# Autodesk Inventor assembly: elric20
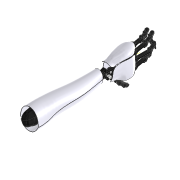
[picture p0: Inventor's stored thumbnail of the model, 180x180]
Saved by Autodesk Inventor 2020.2 (Build 242310000, 310)
## iProperties
Created: 2020-04-12
Part Number: elric20
Document SubType Name: Assembly
Designer: Bardo91
Author: Bardo91
## Documents named in this file (5)
- D:\programming\bioarm\hardware\elric20.iam
- D:\programming\bioarm\hardware\1. hand\elric20-01A.iam
- D:\programming\bioarm\hardware\2. arm\elric20-02A.iam
- D:\programming\bioarm\hardware\2. arm\case\arm_case_1.ipt
- D:\programming\bioarm\hardware\2. arm\case\arm_case_2.ipt
## Components (4 placed, 4 different names)
1. elric20-01A:1 [sub-assembly] — Mate:1, Mate:2
2. elric20-02A:1 [sub-assembly] — Mate:1, Mate:2
3. arm_case_1:1 — Flush:1, Flush:2, Flush:3
4. arm_case_2:1 — Flush:1, Flush:2, Flush:3
## Relationships (5: Flush 3, Mate 2)
- Mate:1: elric20-01A:1 ↔ elric20-02A:1
- Mate:2 (0.5 mm): elric20-01A:1 ↔ elric20-02A:1
- Flush:1: arm_case_1:1 ↔ arm_case_2:1
- Flush:2: arm_case_1:1 ↔ arm_case_2:1
- Flush:3: arm_case_1:1 ↔ arm_case_2:1
